# Autodesk Inventor assembly: robot
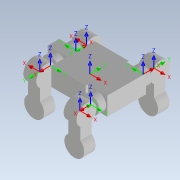
[picture p0: Inventor's stored thumbnail of the model, 180x180]
Saved by Autodesk Inventor 2020 (Build 240168000, 168)
## iProperties
Created: 2021-01-29
Part Number: robot
Document SubType Name: Assembly
Designer: DELL
Author: DELL
## Documents named in this file (4)
- F:\SoftRobot2.0\FlexipodHardware2.0\FlexipodHardware\Flexipod2.0\Cadquery_module\v8.0\robot.iam
- F:\SoftRobot2.0\FlexipodHardware2.0\FlexipodHardware\Flexipod2.0\Cadquery_module\v8.0\body.ipt
- F:\SoftRobot2.0\FlexipodHardware2.0\FlexipodHardware\Flexipod2.0\Cadquery_module\v8.0\hip.ipt
- F:\SoftRobot2.0\FlexipodHardware2.0\FlexipodHardware\Flexipod2.0\Cadquery_module\v8.0\thigh.ipt
## Components (9 placed, 3 different names)
1. body:1 — Flush:1, Flush:2, Flush:3, Mate:1, Mate:2, Mate:3, Mate:4, Mate:5, Mate:6, Mate:7, Mate:8, Angle:1, Angle:2, Angle:3, Angle:4, Angle:5, Angle:6, Angle:7, Angle:8
2. hip:1 — Mate:3, Mate:4, Angle:2, Mate:10, Mate:14
3. hip:2 — Mate:1, Mate:2, Angle:1, Mate:9, Flush:4
4. hip:3 — Mate:7, Mate:8, Angle:4, Mate:12, Flush:5
5. hip:4 — Mate:5, Mate:6, Angle:3, Mate:11, Mate:13
6. thigh:1 — Mate:9, Flush:4, Angle:7
7. thigh:2 — Mate:10, Mate:14, Angle:5
8. thigh:3 — Mate:11, Mate:13, Angle:8
9. thigh:4 — Mate:12, Flush:5, Angle:6
## Relationships (27: Mate 14, Angle 8, Flush 5)
- Flush:1: body:1
- Flush:2: body:1
- Flush:3: body:1
- Mate:1: body:1 ↔ hip:2
- Mate:2: body:1 ↔ hip:2
- Mate:3: body:1 ↔ hip:1
- Mate:4: body:1 ↔ hip:1
- Mate:5: body:1 ↔ hip:4
- Mate:6: body:1 ↔ hip:4
- Mate:7: body:1 ↔ hip:3
- Mate:8: body:1 ↔ hip:3
- Angle:1 (0 deg): body:1 ↔ hip:2
- Angle:2 (0 deg): body:1 ↔ hip:1
- Angle:3 (0 deg): body:1 ↔ hip:4
- Angle:4 (0 deg): body:1 ↔ hip:3
- Mate:9: hip:2 ↔ thigh:1
- Mate:10: hip:1 ↔ thigh:2
- Mate:11: hip:4 ↔ thigh:3
- Mate:12: hip:3 ↔ thigh:4
- Flush:4: hip:2 ↔ thigh:1
- Mate:13: hip:4 ↔ thigh:3
- Flush:5: hip:3 ↔ thigh:4
- Mate:14: hip:1 ↔ thigh:2
- Angle:5 (0 deg): body:1 ↔ thigh:2
- Angle:6 (0 deg): body:1 ↔ thigh:4
- Angle:7 (0 deg): body:1 ↔ thigh:1
- Angle:8 (0 deg): body:1 ↔ thigh:3
